# Autodesk Inventor assembly: Pulley
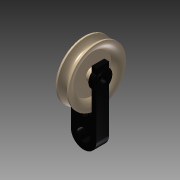
[picture p0: Inventor's stored thumbnail of the model, 180x180]
Saved by Autodesk Inventor 2014 (Build 180170000, 170)
## iProperties
Created: 2013-10-13
Part Number: Pulley
Document SubType Name: Assembly
Designer: david
Author: david
## Documents named in this file (3)
- C:\Users\david\Documents\Pulley.iam
- C:\Users\david\Documents\pulley wheel.ipt
- C:\Users\david\Documents\pulley hook.ipt
## Components (2 placed, 2 different names)
1. pulley wheel:1 — Rotational:1
2. pulley hook:1 — Rotational:1
## Relationships (1: RevoluteJoint 1)
- Rotational:1 [RevoluteJoint]: pulley wheel:1 ↔ pulley hook:1
